# Autodesk Inventor assembly: Assembly
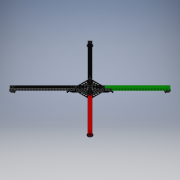
[picture p0: Inventor's stored thumbnail of the model, 180x180]
Saved by Autodesk Inventor 2016 (Build 200138000, 138)
## iProperties
Created: 2016-03-06
Part Number: Assembly
Document SubType Name: Assembly
Designer: dimas
Author: dimas
## Documents named in this file (5)
- C:\Users\dimas\Documents\lap_quad\Assembly.iam
- C:\Users\dimas\Documents\lap_quad\Arm_light.ipt
- C:\Users\dimas\Documents\lap_quad\frame_mount.ipt
- C:\Users\dimas\Documents\lap_quad\plate_mk2.ipt
- C:\Users\dimas\Documents\lap_quad\motor_mount.ipt
## Components (14 placed, 4 different names)
1. Arm_light:1 — Mate:1, Mate:2, Flush:1, Mate:25, Mate:26, Mate:27
2. frame_mount:1 — Mate:1, Mate:2, Flush:1, Mate:3, Mate:4, Flush:2, Mate:5, Mate:6, Flush:3
3. plate_mk2:1 — Mate:3, Mate:4, Flush:2, Mate:7, Mate:8, Mate:9, Mate:10, Mate:11, Mate:12, Mate:13, Mate:14, Mate:15, Flush:7, Flush:8, Flush:9
4. plate_mk2:2 — Mate:5, Mate:6, Flush:3
5. frame_mount:2 — Mate:7, Mate:8, Mate:9, Mate:16, Mate:17, Flush:4
6. frame_mount:3 — Mate:13, Mate:14, Mate:15, Mate:20, Mate:21, Flush:6
7. frame_mount:4 — Mate:10, Mate:11, Mate:12, Mate:18, Mate:19, Flush:5
8. Arm_light:2 — Mate:16, Mate:17, Flush:4, Mate:28, Mate:29, Mate:30
9. Arm_light:3 — Mate:18, Mate:19, Flush:5, Mate:31, Mate:32, Mate:33
10. Arm_light:4 — Mate:20, Mate:21, Flush:6, Mate:22, Mate:23, Mate:24
11. motor_mount:1 — Mate:22, Mate:23, Mate:24
12. motor_mount:2 — Mate:25, Mate:26, Mate:27
13. motor_mount:3 — Mate:28, Mate:29, Mate:30
14. motor_mount:4 — Mate:31, Mate:32, Mate:33
## Relationships (42: Mate 33, Flush 9)
- Mate:1: Arm_light:1 ↔ frame_mount:1
- Mate:2: Arm_light:1 ↔ frame_mount:1
- Flush:1: Arm_light:1 ↔ frame_mount:1
- Mate:3: frame_mount:1 ↔ plate_mk2:1
- Mate:4: frame_mount:1 ↔ plate_mk2:1
- Flush:2: frame_mount:1 ↔ plate_mk2:1
- Mate:5: frame_mount:1 ↔ plate_mk2:2
- Mate:6: frame_mount:1 ↔ plate_mk2:2
- Flush:3: frame_mount:1 ↔ plate_mk2:2
- Mate:7: plate_mk2:1 ↔ frame_mount:2
- Mate:8: plate_mk2:1 ↔ frame_mount:2
- Mate:9: plate_mk2:1 ↔ frame_mount:2
- Mate:10: plate_mk2:1 ↔ frame_mount:4
- Mate:11: plate_mk2:1 ↔ frame_mount:4
- Mate:12: plate_mk2:1 ↔ frame_mount:4
- Mate:13: plate_mk2:1 ↔ frame_mount:3
- Mate:14: plate_mk2:1 ↔ frame_mount:3
- Mate:15: plate_mk2:1 ↔ frame_mount:3
- Mate:16: frame_mount:2 ↔ Arm_light:2
- Mate:17: frame_mount:2 ↔ Arm_light:2
- Flush:4: frame_mount:2 ↔ Arm_light:2
- Mate:18: frame_mount:4 ↔ Arm_light:3
- Mate:19: frame_mount:4 ↔ Arm_light:3
- Flush:5: frame_mount:4 ↔ Arm_light:3
- Mate:20: frame_mount:3 ↔ Arm_light:4
- Mate:21: frame_mount:3 ↔ Arm_light:4
- Flush:6: frame_mount:3 ↔ Arm_light:4
- Flush:7: plate_mk2:1
- Flush:8: plate_mk2:1
- Flush:9: plate_mk2:1
- Mate:22: Arm_light:4 ↔ motor_mount:1
- Mate:23: Arm_light:4 ↔ motor_mount:1
- Mate:24: Arm_light:4 ↔ motor_mount:1
- Mate:25: Arm_light:1 ↔ motor_mount:2
- Mate:26: Arm_light:1 ↔ motor_mount:2
- Mate:27: Arm_light:1 ↔ motor_mount:2
- Mate:28: Arm_light:2 ↔ motor_mount:3
- Mate:29: Arm_light:2 ↔ motor_mount:3
- Mate:30: Arm_light:2 ↔ motor_mount:3
- Mate:31: Arm_light:3 ↔ motor_mount:4
- Mate:32: Arm_light:3 ↔ motor_mount:4
- Mate:33: Arm_light:3 ↔ motor_mount:4
